# Autodesk Inventor assembly: 4Wire-FDM-Slot
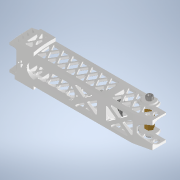
[picture p0: Inventor's stored thumbnail of the model, 180x180]
Saved by Autodesk Inventor 2021 (Build 250183000, 183)
## iProperties
Created: 2020-08-18
Part Number: 4Wire-FDM-Slot
Document SubType Name: Assembly
Designer: lucas
Author: lucas
## Documents named in this file (6)
- C:\Users\lucas\Nextcloud\HackerSpace\HV Home Battery Storage Project\Concepts & Storyboards\18650 4wire Holder\4Wire-FDM-Slot\4Wire-FDM-Slot.iam
- C:\Users\lucas\Nextcloud\HackerSpace\HV Home Battery Storage Project\Concepts & Storyboards\18650 4wire Holder\4Wire-FDM-Slot\FDM-Slot.ipt
- C:\Users\lucas\Nextcloud\HackerSpace\HV Home Battery Storage Project\Concepts & Storyboards\18650 4wire Holder\4Wire-FDM-Slot\Standoff-M3x20mm.ipt
- C:\Users\lucas\Nextcloud\HackerSpace\HV Home Battery Storage Project\Concepts & Storyboards\18650 4wire Holder\ZKE\ZKE-Term-Sprung-17.5mm.ipt
- C:\Users\lucas\Documents\Inventor\Content Center Files\R2021\en-US\ISO 4762(2)\ISO 4762 - M3 x 6ISO.ipt
- C:\Users\lucas\Nextcloud\HackerSpace\HV Home Battery Storage Project\Concepts & Storyboards\18650 4wire Holder\Shared Parts\Pogo_pin_P75-E2.ipt
## Components (6 placed, 5 different names)
1. FDM-Slot:1 — Rotational:1, Rigid:1, Mate:1, Mate:2, Insert:1
2. Shaft:1 — Rotational:1
3. ZKE-Term-Sprung-17.5mm:1 — Rigid:1, Rigid:2
4. ISO 4762 M3 x 6:1 — Mate:1, Mate:2
5. ISO 4762 M3 x 6:2 — Insert:1
6. Pogo_pin_P75-E2:1 — Rigid:2
## Relationships (6: WeldJoint 2, Mate 2, RevoluteJoint 1, Insert 1)
- Rotational:1 [RevoluteJoint]: FDM-Slot:1 ↔ Shaft:1
- Rigid:1 [WeldJoint]: FDM-Slot:1 ↔ ZKE-Term-Sprung-17.5mm:1
- Mate:1: FDM-Slot:1 ↔ ISO 4762 M3 x 6:1
- Mate:2: FDM-Slot:1 ↔ ISO 4762 M3 x 6:1
- Insert:1: FDM-Slot:1 ↔ ISO 4762 M3 x 6:2
- Rigid:2 [WeldJoint]: ZKE-Term-Sprung-17.5mm:1 ↔ Pogo_pin_P75-E2:1
